# Autodesk Inventor assembly: SC-6-F
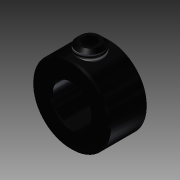
[picture p0: Inventor's stored thumbnail of the model, 180x180]
Saved by Autodesk Inventor 2014 (Build 180170000, 170)
## iProperties
Category: Miscellaneous
Company: Autodesk Inc.
Created: 2013-12-18
Part Number: SC-6-F
Document SubType Name: Assembly
Designer: Autodesk Inc.
Catalog Web Link: http://www.ruland.com/shaft-collar.php?recordID=SC-6-F
Description: 3/8" ID 3/4" OD shaft collar
Vendor: Ruland Manufacturing
Author: Autodesk Inc.
## Documents named in this file (3)
- D:\Data Folder\FIRST 2014\KOP Parts\Miscellaneous\MISC_ShaftCollar_SC-6-F.iam
- D:\Data Folder\FIRST 2014\KOP Parts\Miscellaneous\MISC_ShaftCollar_SC-6-F.ipt
- D:\Data Folder\FIRST 2014\KOP Parts\Miscellaneous\ANSI B18.3 - 1_4-20 UNC - 0.25(24).ipt
## Components (2 placed, 2 different names)
1. MISC_ShaftCollar_SC-6-F:1 — Mate:1
2. Hexagon Socket Set Screw - Flat Point - Inch 1/4-20 UNC x 0.25:1 — Mate:1, Flush:1
## Relationships (2: Mate 1, Flush 1)
- Mate:1: MISC_ShaftCollar_SC-6-F:1 ↔ Hexagon Socket Set Screw - Flat Point - Inch 1/4-20 UNC x 0.25:1
- Flush:1 (-11.43 mm): Hexagon Socket Set Screw - Flat Point - Inch 1/4-20 UNC x 0.25:1
